# Autodesk Inventor assembly: assembly
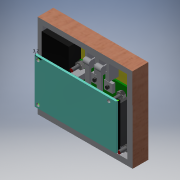
[picture p0: Inventor's stored thumbnail of the model, 180x180]
Saved by Autodesk Inventor 2017 (Build 210142000, 142)
## iProperties
Created: 2016-11-05
Part Number: assembly
Document SubType Name: Assembly
Designer: radrajith
Author: radrajith
## Documents named in this file (7)
- C:\Users\radra\Box Sync\Senior Fall 2016\ESE 323\autocad\assembly.iam
- C:\Users\radra\Box Sync\Senior Fall 2016\ESE 323\autocad\lab 04.ipt
- C:\Users\radra\Box Sync\Senior Fall 2016\ESE 323\autocad\battery.ipt
- C:\Users\radra\Documents\Inventor\Content Center Files\R2017\en-US\ANSI B18.2.4.2M\ANSI B18.2.4.2M - M3.5x0.6 - 6.ipt
- C:\Users\radra\Box Sync\Senior Fall 2016\ESE 323\autocad\lcd display.ipt
- C:\Users\radra\Box Sync\Senior Fall 2016\ESE 323\autocad\case_bottom_new.ipt
- C:\Users\radra\Box Sync\Senior Fall 2016\ESE 323\autocad\button_press_new.ipt
## Components (9 placed, 6 different names)
1. lab 04:1 — Insert:1, Insert:5, Mate:2, Mate:4, Mate:6, Mate:16
2. case_bottom_new:1 — Insert:1, Insert:5, Mate:1, Mate:3, Mate:5, Mate:13, Mate:14, Mate:15
3. battery:1 — Mate:13, Mate:14, Mate:15
4. button_press_new:2
5. button_press_new:1
6. ANSI B18.2.4.2M M3.5x0.6:1 — Mate:1, Mate:2
7. ANSI B18.2.4.2M M3.5x0.6:2 — Mate:3, Mate:4
8. ANSI B18.2.4.2M M3.5x0.6:3 — Mate:5, Mate:6
9. lcd display:1 — Mate:16
## Relationships (18: Mate 16, Insert 2)
- Insert:1 (10 mm): lab 04:1 ↔ case_bottom_new:1
- Insert:5 (10 mm): lab 04:1 ↔ case_bottom_new:1
- Mate:1: case_bottom_new:1 ↔ ANSI B18.2.4.2M M3.5x0.6:1
- Mate:2: lab 04:1 ↔ ANSI B18.2.4.2M M3.5x0.6:1
- Mate:3: case_bottom_new:1 ↔ ANSI B18.2.4.2M M3.5x0.6:2
- Mate:4: lab 04:1 ↔ ANSI B18.2.4.2M M3.5x0.6:2
- Mate:5: case_bottom_new:1 ↔ ANSI B18.2.4.2M M3.5x0.6:3
- Mate:6: lab 04:1 ↔ ANSI B18.2.4.2M M3.5x0.6:3
- [Mate]: lab 04:1 ↔ button_press_new:1
- [Mate]: case_bottom_new:1 ↔ button_press_new:1
- [Mate]: case_bottom_new:1 ↔ button_press_new:1
- [Mate]: lab 04:1 ↔ button_press_new:2
- [Mate]: case_bottom_new:1 ↔ button_press_new:2
- [Mate]: case_bottom_new:1 ↔ button_press_new:2
- Mate:13: case_bottom_new:1 ↔ battery:1
- Mate:14: case_bottom_new:1 ↔ battery:1
- Mate:15: case_bottom_new:1 ↔ battery:1
- Mate:16: lab 04:1 ↔ lcd display:1
